# Autodesk Inventor assembly: Butterfly Drive Module
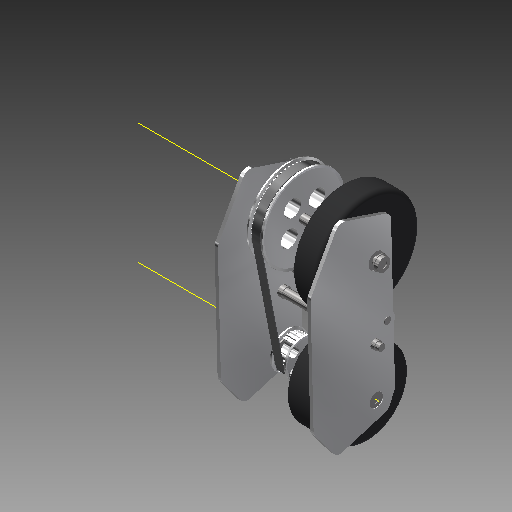
[picture p0: Inventor's stored thumbnail of the model, 512x512]
Saved by Autodesk Inventor 2019 (Build 230136000, 136)
## iProperties
Created: 2019-10-18
Part Number: Butterfly Drive Module
Document SubType Name: Assembly
Designer: admin
Author: admin
## Documents named in this file (11)
- C:\Users\Mark\Desktop\7738 Helion Engineering\7738-CAD-prep\Butterfly drive\Butterfly Drive Module.iam
- C:\Users\Mark\Desktop\7738 Helion Engineering\7738-CAD-prep\Butterfly drive\100mm Mecanum StandIn.ipt
- C:\Users\Mark\Desktop\7738 Helion Engineering\7738-CAD-prep\Butterfly drive\100mm Traction Wheel StandIn.ipt
- C:\Users\Mark\Desktop\7738 Helion Engineering\7738-CAD-prep\Butterfly drive\Butterfly Drive Module\Design Accelerator\Synchronous Belts Transmission3.iam
- C:\Users\Mark\Desktop\7738 Helion Engineering\7738-CAD-prep\Butterfly drive\F688ZZ 8mm ID Flange.ipt
- C:\Users\Mark\Desktop\7738 Helion Engineering\7738-CAD-prep\Butterfly drive\F6800Z 10mm ID Flange.ipt
- C:\Users\Mark\Desktop\7738 Helion Engineering\7738-CAD-prep\Butterfly drive\Mecanum Axle.ipt
- C:\Users\Mark\Desktop\7738 Helion Engineering\7738-CAD-prep\Butterfly drive\Motor Axle.ipt
- C:\Users\Mark\Desktop\7738 Helion Engineering\7738-CAD-prep\Butterfly drive\Module Plate 1.ipt
- C:\Users\Mark\Desktop\7738 Helion Engineering\7738-CAD-prep\Butterfly drive\Module Pneumatic Axle.ipt
- C:\Users\Mark\Desktop\7738 Helion Engineering\7738-CAD-prep\Butterfly drive\Stopper Axle.ipt
## Components (14 placed, 10 different names)
1. 100mm Mecanum StandIn:1 — Flush:1, Mate:5, Mate:7, Angle:1, Mate:8, Mate:13, Mate:16
2. 100mm Traction Wheel StandIn:1 — Mate:4, Flush:1, Mate:6, Mate:14
3. Synchronous Belts Transmission:1 [sub-assembly] — Mate:5, Mate:6, Mate:7, Mate:10, Mate:15
4. F688ZZ 8mm ID Flange:1 — Mate:8, Mate:13, Flush:2, Mate:17, Mate:21, Mate:22
5. F688ZZ 8mm ID Flange:3 — Mate:10, Mate:24, Mate:26
6. F6800Z 10mm ID Flange:1 — Mate:14, Flush:2, Mate:18, Flush:4
7. F6800Z 10mm ID Flange:2 — Mate:15
8. Mecanum Axle:1 — Mate:16, Mate:17
9. F688ZZ 8mm ID Flange:4 — Mate:18, Flush:4, Mate:19, Mate:20
10. Motor Axle:1 — Mate:19, Mate:20
11. Module Plate 1:1 — Mate:21, Mate:22, Mate:23, Mate:29, Mate:31
12. Module Plate 1:2 — Mate:24, Mate:25, Mate:26, Mate:30, Mate:32
13. Module Pneumatic Axle:1 — Mate:29, Mate:30
14. Stopper Axle:1 — Mate:31, Mate:32
## Relationships (28: Mate 24, Flush 3, Angle 1)
- Mate:4: 100mm Traction Wheel StandIn:1
- Flush:1: 100mm Mecanum StandIn:1 ↔ 100mm Traction Wheel StandIn:1
- Mate:5: 100mm Mecanum StandIn:1 ↔ Synchronous Belts Transmission:1
- Mate:6: 100mm Traction Wheel StandIn:1 ↔ Synchronous Belts Transmission:1
- Mate:7 (2 mm): 100mm Mecanum StandIn:1 ↔ Synchronous Belts Transmission:1
- Angle:1 (90 deg): 100mm Mecanum StandIn:1
- Mate:8: 100mm Mecanum StandIn:1 ↔ F688ZZ 8mm ID Flange:1
- Mate:10 (4 mm): Synchronous Belts Transmission:1 ↔ F688ZZ 8mm ID Flange:3
- Mate:13 (5 mm): 100mm Mecanum StandIn:1 ↔ F688ZZ 8mm ID Flange:1
- Mate:14: 100mm Traction Wheel StandIn:1 ↔ F6800Z 10mm ID Flange:1
- Mate:15: Synchronous Belts Transmission:1 ↔ F6800Z 10mm ID Flange:2
- Flush:2: F688ZZ 8mm ID Flange:1 ↔ F6800Z 10mm ID Flange:1
- Mate:16: 100mm Mecanum StandIn:1 ↔ Mecanum Axle:1
- Mate:17 (0.3 mm): F688ZZ 8mm ID Flange:1 ↔ Mecanum Axle:1
- Mate:18: F6800Z 10mm ID Flange:1 ↔ F688ZZ 8mm ID Flange:4
- Flush:4 (-9.3 mm): F6800Z 10mm ID Flange:1 ↔ F688ZZ 8mm ID Flange:4
- Mate:19 (0.3 mm): F688ZZ 8mm ID Flange:4 ↔ Motor Axle:1
- Mate:20: F688ZZ 8mm ID Flange:4 ↔ Motor Axle:1
- Mate:21: F688ZZ 8mm ID Flange:1 ↔ Module Plate 1:1
- Mate:22 (0.3 mm): F688ZZ 8mm ID Flange:1 ↔ Module Plate 1:1
- Mate:23: Module Plate 1:1
- Mate:24: F688ZZ 8mm ID Flange:3 ↔ Module Plate 1:2
- Mate:25: Module Plate 1:2
- Mate:26 (0.3 mm): F688ZZ 8mm ID Flange:3 ↔ Module Plate 1:2
- Mate:29 (0.3 mm): Module Plate 1:1 ↔ Module Pneumatic Axle:1
- Mate:30: Module Plate 1:2 ↔ Module Pneumatic Axle:1
- Mate:31: Module Plate 1:1 ↔ Stopper Axle:1
- Mate:32 (0.3 mm): Module Plate 1:2 ↔ Stopper Axle:1
